# Autodesk Inventor assembly: Robot
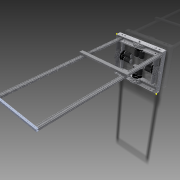
[picture p0: Inventor's stored thumbnail of the model, 180x180]
Saved by Autodesk Inventor 2015 (Build 190159000, 159)
## iProperties
Created: 2015-01-10
Part Number: Robot
Document SubType Name: Assembly
Designer: jhirshland1
Author: jhirshland1
## Documents named in this file (7)
- C:\Users\jhirshland1\Inventor\HWRobot2015CAD\Chassis\Chassis.iam
- C:\Users\jhirshland1\Inventor\HWRobot2015CAD\FRCKOP2015\Drive Base\am-2951 AM14U2 Outside Sheet.ipt
- C:\Users\jhirshland1\Inventor\HWRobot2015CAD\FRCKOP2015\Drive Base\am-2951 AM14U2 Ouside 23i.ipt
- C:\Users\jhirshland1\Inventor\HWRobot2015CAD\FRCKOP2015\Drive Base\am-2952 AM14U2 Inside Sheet.ipt
- C:\Users\jhirshland1\Inventor\HWRobot2015CAD\FRCKOP2015\AndyMark\WheelAssembly.iam
- C:\Users\jhirshland1\Inventor\HWRobot2015CAD\FRCKOP2015\AndyMark\SecondWheelAssembl.iam
- C:\Users\jhirshland1\Inventor\HWRobot2015CAD\Elevator\Elevator.iam
## Components (11 placed, 6 different names)
1. am-2951 AM14U2 Outside Sheet:1 — Mate:5, Mate:8
2. am-2951 AM14U2 Outside Sheet:2 — Mate:22, Flush:13, Flush:14
3. am-2951 AM14U2 Ouside 23i:1 — Mate:5, Mate:19
4. am-2951 AM14U2 Ouside 23i:2 — Mate:8, Mate:13, Mate:17, Mate:21, Mate:22, Flush:13, Flush:14
5. am-2952 AM14U2 Inside Sheet:1 — Mate:17, Mate:18, Mate:20, Flush:11, Flush:12, Mate:23, Mate:24
6. am-2952 AM14U2 Inside Sheet:2 — Mate:13, Insert:3, Insert:4
7. WheelAssembly:1 [sub-assembly]
8. WheelAssembly:2 [sub-assembly] — Insert:3, Insert:4
9. SecondWheelAssembl:1 [sub-assembly] — Mate:18, Mate:19, Flush:12
10. SecondWheelAssembl:2 [sub-assembly] — Mate:20, Flush:11, Mate:21
11. Elevator:1 [sub-assembly] — Mate:23, Mate:24
## Relationships (19: Mate 11, Insert 4, Flush 4)
- Mate:5: am-2951 AM14U2 Outside Sheet:1 ↔ am-2951 AM14U2 Ouside 23i:1
- Mate:8: am-2951 AM14U2 Outside Sheet:1 ↔ am-2951 AM14U2 Ouside 23i:2
- Mate:13: am-2951 AM14U2 Ouside 23i:2 ↔ am-2952 AM14U2 Inside Sheet:2
- Mate:17: am-2951 AM14U2 Ouside 23i:2 ↔ am-2952 AM14U2 Inside Sheet:1
- [Insert]: am-2952 AM14U2 Inside Sheet:1 ↔ WheelAssembly:1
- [Insert]: am-2952 AM14U2 Inside Sheet:1 ↔ WheelAssembly:1
- Insert:3: am-2952 AM14U2 Inside Sheet:2 ↔ WheelAssembly:2
- Insert:4: am-2952 AM14U2 Inside Sheet:2 ↔ WheelAssembly:2
- Mate:18: am-2952 AM14U2 Inside Sheet:1 ↔ SecondWheelAssembl:1
- Mate:19 (85.09 mm): am-2951 AM14U2 Ouside 23i:1 ↔ SecondWheelAssembl:1
- Mate:20: am-2952 AM14U2 Inside Sheet:1 ↔ SecondWheelAssembl:2
- Flush:11: am-2952 AM14U2 Inside Sheet:1 ↔ SecondWheelAssembl:2
- Mate:21 (85.09 mm): am-2951 AM14U2 Ouside 23i:2 ↔ SecondWheelAssembl:2
- Flush:12: am-2952 AM14U2 Inside Sheet:1 ↔ SecondWheelAssembl:1
- Mate:22: am-2951 AM14U2 Outside Sheet:2 ↔ am-2951 AM14U2 Ouside 23i:2
- Flush:13: am-2951 AM14U2 Outside Sheet:2 ↔ am-2951 AM14U2 Ouside 23i:2
- Flush:14: am-2951 AM14U2 Outside Sheet:2 ↔ am-2951 AM14U2 Ouside 23i:2
- Mate:23: am-2952 AM14U2 Inside Sheet:1 ↔ Elevator:1
- Mate:24: am-2952 AM14U2 Inside Sheet:1 ↔ Elevator:1
